# Autodesk Inventor assembly: Final_Assembly
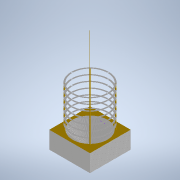
[picture p0: Inventor's stored thumbnail of the model, 180x180]
Saved by Autodesk Inventor 2021 (Build 250183000, 183)
## iProperties
Created: 2020-07-14
Part Number: Final_Assembly
Document SubType Name: Assembly
Designer: aydan
Author: aydan
## Documents named in this file (4)
- C:\Users\aydan\OneDrive\Documents\Inventor\Garcia_Lab\Final_Assembly.iam
- C:\Users\aydan\OneDrive\Documents\Inventor\Garcia_Lab\RF_Funnel\funnel.iam
- C:\Users\aydan\OneDrive\Documents\Inventor\Garcia_Lab\DC_Cage\DC_Cage.iam
- C:\Users\aydan\OneDrive\Documents\Inventor\Garcia_Lab\DC_Cage\cage_electrode.ipt
## Components (9 placed, 3 different names)
1. funnel:1 [sub-assembly] — Mate:1, Flush:1, Flush:2, Mate:2
2. DC_Cage:1 [sub-assembly] — Mate:1, Flush:1, Flush:2, Mate:2, Mate:5, Mate:7, Mate:9, Mate:11, Mate:13, Mate:16, Mate:17, Mate:19, Mate:21
3. cage_electrode:1 — Mate:6, Mate:7
4. cage_electrode:2 — Mate:8, Mate:9
5. cage_electrode:3 — Mate:15, Mate:17
6. cage_electrode:4 — Mate:10, Mate:11
7. cage_electrode:5 — Mate:12, Mate:13
8. cage_electrode:7 — Mate:14, Mate:16
9. cage_electrode:8 — Mate:18, Mate:19
## Relationships (20: Mate 18, Flush 2)
- Mate:1: funnel:1 ↔ DC_Cage:1
- Flush:1: funnel:1 ↔ DC_Cage:1
- Flush:2: funnel:1 ↔ DC_Cage:1
- Mate:2: funnel:1 ↔ DC_Cage:1
- Mate:5: DC_Cage:1
- Mate:6: cage_electrode:1
- Mate:7 (9.9 mm): DC_Cage:1 ↔ cage_electrode:1
- Mate:8: cage_electrode:2
- Mate:9 (19.9 mm): DC_Cage:1 ↔ cage_electrode:2
- Mate:10: cage_electrode:4
- Mate:11 (29.9 mm): DC_Cage:1 ↔ cage_electrode:4
- Mate:12: cage_electrode:5
- Mate:13 (39.9 mm): DC_Cage:1 ↔ cage_electrode:5
- Mate:14: cage_electrode:7
- Mate:15: cage_electrode:3
- Mate:16 (49.9 mm): DC_Cage:1 ↔ cage_electrode:7
- Mate:17 (59.9 mm): DC_Cage:1 ↔ cage_electrode:3
- Mate:18: cage_electrode:8
- Mate:19 (69.9 mm): DC_Cage:1 ↔ cage_electrode:8
- Mate:21: DC_Cage:1
